# Autodesk Inventor assembly: mg996r_top
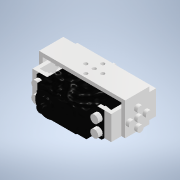
[picture p0: Inventor's stored thumbnail of the model, 180x180]
Saved by Autodesk Inventor 2021.4 (Build 254397000, 397)
## iProperties
Created: 2022-07-24
Part Number: mg996r_top
Document SubType Name: Assembly
Designer: isamu
Author: isamu
## Documents named in this file (5)
- D:\personal_projects\robot\inventor\2021_matlab_compat\mg996r_top.iam
- D:\personal_projects\robot\inventor\2021_matlab_compat\mg996r_servo_frame_with_axis.iam
- D:\personal_projects\robot\exports\frames\servo frame part 3.ipt
- D:\personal_projects\robot\exports\screws\m3 nuts.ipt
- D:\personal_projects\robot\exports\screws\m3x8.ipt
## Components (22 placed, 4 different names)
1. mg996r_servo_frame_with_axis:1 [sub-assembly] — Mate:1, Mate:2, Mate:3, Insert:11, Insert:12, Insert:13, Insert:14, Insert:15, Insert:16, Insert:17, Insert:18, Insert:19, Insert:20
2. servo frame part 3:1 — Mate:1, Mate:2, Mate:3, Insert:1, Insert:2, Insert:3, Insert:4, Insert:5, Insert:6, Insert:7, Insert:8, Insert:9, Insert:10
3. m3 nuts:1 — Insert:15
4. m3 nuts:2 — Insert:13
5. m3 nuts:3 — Insert:12
6. m3 nuts:4 — Insert:11
7. m3 nuts:5 — Insert:14
8. m3 nuts:6 — Insert:20
9. m3 nuts:7 — Insert:19
10. m3 nuts:8 — Insert:18
11. m3 nuts:9 — Insert:17
12. m3 nuts:10 — Insert:16
13. m3x8:1 — Insert:10
14. m3x8:2 — Insert:1
15. m3x8:3 — Insert:7
16. m3x8:4 — Insert:9
17. m3x8:5 — Insert:8
18. m3x8:6 — Insert:2
19. m3x8:7 — Insert:3
20. m3x8:8 — Insert:4
21. m3x8:9 — Insert:5
22. m3x8:10 — Insert:6
## Relationships (23: Insert 20, Mate 3)
- Mate:1: mg996r_servo_frame_with_axis:1 ↔ servo frame part 3:1
- Mate:2: mg996r_servo_frame_with_axis:1 ↔ servo frame part 3:1
- Mate:3: mg996r_servo_frame_with_axis:1 ↔ servo frame part 3:1
- Insert:1: servo frame part 3:1 ↔ m3x8:2
- Insert:2: servo frame part 3:1 ↔ m3x8:6
- Insert:3: servo frame part 3:1 ↔ m3x8:7
- Insert:4: servo frame part 3:1 ↔ m3x8:8
- Insert:5: servo frame part 3:1 ↔ m3x8:9
- Insert:6: servo frame part 3:1 ↔ m3x8:10
- Insert:7: servo frame part 3:1 ↔ m3x8:3
- Insert:8: servo frame part 3:1 ↔ m3x8:5
- Insert:9: servo frame part 3:1 ↔ m3x8:4
- Insert:10: servo frame part 3:1 ↔ m3x8:1
- Insert:11: mg996r_servo_frame_with_axis:1 ↔ m3 nuts:4
- Insert:12: mg996r_servo_frame_with_axis:1 ↔ m3 nuts:3
- Insert:13: mg996r_servo_frame_with_axis:1 ↔ m3 nuts:2
- Insert:14: mg996r_servo_frame_with_axis:1 ↔ m3 nuts:5
- Insert:15: mg996r_servo_frame_with_axis:1 ↔ m3 nuts:1
- Insert:16: mg996r_servo_frame_with_axis:1 ↔ m3 nuts:10
- Insert:17: mg996r_servo_frame_with_axis:1 ↔ m3 nuts:9
- Insert:18: mg996r_servo_frame_with_axis:1 ↔ m3 nuts:8
- Insert:19: mg996r_servo_frame_with_axis:1 ↔ m3 nuts:7
- Insert:20: mg996r_servo_frame_with_axis:1 ↔ m3 nuts:6
